# Autodesk Inventor assembly: finalassy
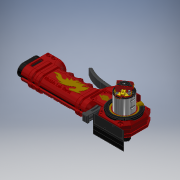
[picture p0: Inventor's stored thumbnail of the model, 180x180]
Saved by Autodesk Inventor 2018 (Build 220112000, 112)
## iProperties
Created: 2019-02-22
Part Number: finalassy
Material: 一般
Document SubType Name: Assembly
Designer: ku_sk
Author: ku_sk
## Documents named in this file (22)
- D:\Inventor\BayBladeLauncher\finalassy.iam
- D:\Inventor\BayBladeLauncher\parts\battery.ipt
- D:\Inventor\BayBladeLauncher\parts\brake.ipt
- D:\Inventor\BayBladeLauncher\parts\bay conect.ipt
- D:\Inventor\BayBladeLauncher\parts\bearing.ipt
- D:\Inventor\BayBladeLauncher\parts\bar.ipt
- D:\Inventor\BayBladeLauncher\parts\topcover.ipt
- D:\Inventor\BayBladeLauncher\parts\bar2.ipt
- D:\Inventor\BayBladeLauncher\parts\joint.ipt
- D:\Inventor\BayBladeLauncher\parts\switch.ipt
- D:\Inventor\BayBladeLauncher\parts\cover.ipt
- D:\Inventor\BayBladeLauncher\parts\ring.ipt
- D:\Inventor\BayBladeLauncher\parts\circuitcover.ipt
- D:\Inventor\BayBladeLauncher\parts\circuitcover1.ipt
- D:\Inventor\BayBladeLauncher\parts\gear.ipt
- D:\Inventor\BayBladeLauncher\parts\dragon.ipt
- D:\Inventor\BayBladeLauncher\parts\dragon_MIR.ipt
- D:\Inventor\BayBladeLauncher\parts\skyrimlogo2_1_9.ipt
- D:\Inventor\BayBladeLauncher\parts\pushbar.ipt
- D:\Inventor\BayBladeLauncher\reedy_540_rc_motor-1.snapshot.2\motor.iam
- D:\Inventor\BayBladeLauncher\parts\undercover1.ipt
- D:\Inventor\BayBladeLauncher\parts\undercover2.ipt
## Components (24 placed, 21 different names)
1. battery:1
2. bay conect:1 — メイト:8, メイト:9, メイト:10, メイト:19, フラッシュ:2
3. gear:1 — メイト:40, フラッシュ:2
4. bearing:1 — メイト:8, メイト:9, メイト:20
5. bar:1 — メイト:10, メイト:17, メイト:21, メイト:23, メイト:26
6. topcover:1 — メイト:28, メイト:29, メイト:30, メイト:31, メイト:32, メイト:40, メイト:49, 角度:1, メイト:50, メイト:53, メイト:54, メイト:55
7. bar2:1 — メイト:19, メイト:20, メイト:21
8. joint:1 — メイト:23, メイト:24, メイト:25, メイト:26
9. switch:1 — メイト:24, メイト:25, メイト:51, フラッシュ:4, メイト:52
10. cover:1 — メイト:30, メイト:31, メイト:32
11. ring:1 — メイト:28, メイト:29
12. circuitcover:1 — メイト:36, メイト:37, メイト:38, メイト:39
13. circuitcover1:1 — メイト:36, メイト:37, メイト:38, メイト:39
14. dragon:1
15. dragon_MIR:1
16. skyrimlogo2_1_9:1 — メイト:49, 角度:1, メイト:50
17. pushbar:1 — メイト:51, フラッシュ:4, メイト:52
18. motor:1 [sub-assembly] — メイト:53, メイト:54, メイト:55
19. undercover1:1 — メイト:56, メイト:57, メイト:58, メイト:59, メイト:60, メイト:61, メイト:62, メイト:63, メイト:64
20. undercover2:1 — メイト:56, メイト:57, メイト:58, メイト:59, メイト:60, メイト:61
21. brake:1 — メイト:17
22. brake:2
23. brake:3
24. brake:4
## Component patterns: (4 elements, first: brake:1)
## Relationships (40: Mate 37, Flush 2, Angle 1)
- メイト:8 [Mate]: bay conect:1 ↔ bearing:1
- メイト:9 [Mate]: bay conect:1 ↔ bearing:1
- メイト:10 [Mate]: bay conect:1 ↔ bar:1
- メイト:17 [Mate]: bar:1 ↔ brake:1
- メイト:19 [Mate]: bay conect:1 ↔ bar2:1
- メイト:20 [Mate]: bearing:1 ↔ bar2:1
- メイト:21 [Mate]: bar:1 ↔ bar2:1
- メイト:23 [Mate]: bar:1 ↔ joint:1
- メイト:24 [Mate]: joint:1 ↔ switch:1
- メイト:25 [Mate] (0.25 mm): joint:1 ↔ switch:1
- メイト:26 [Mate]: bar:1 ↔ joint:1
- メイト:28 [Mate]: topcover:1 ↔ ring:1
- メイト:29 [Mate]: topcover:1 ↔ ring:1
- メイト:30 [Mate]: topcover:1 ↔ cover:1
- メイト:31 [Mate]: topcover:1 ↔ cover:1
- メイト:32 [Mate]: topcover:1 ↔ cover:1
- メイト:36 [Mate]: circuitcover:1 ↔ circuitcover1:1
- メイト:37 [Mate]: circuitcover:1 ↔ circuitcover1:1
- メイト:38 [Mate]: circuitcover:1 ↔ circuitcover1:1
- メイト:39 [Mate]: circuitcover:1 ↔ circuitcover1:1
- メイト:40 [Mate]: gear:1 ↔ topcover:1
- フラッシュ:2 [Flush]: bay conect:1 ↔ gear:1
- メイト:49 [Mate]: topcover:1 ↔ skyrimlogo2_1_9:1
- 角度:1 [Angle] (26.37 deg): topcover:1 ↔ skyrimlogo2_1_9:1
- メイト:50 [Mate]: topcover:1 ↔ skyrimlogo2_1_9:1
- メイト:51 [Mate]: switch:1 ↔ pushbar:1
- フラッシュ:4 [Flush]: switch:1 ↔ pushbar:1
- メイト:52 [Mate]: switch:1 ↔ pushbar:1
- メイト:53 [Mate]: topcover:1 ↔ motor:1
- メイト:54 [Mate]: topcover:1 ↔ motor:1
- メイト:55 [Mate]: topcover:1 ↔ motor:1
- メイト:56 [Mate]: undercover1:1 ↔ undercover2:1
- メイト:57 [Mate]: undercover1:1 ↔ undercover2:1
- メイト:58 [Mate]: undercover1:1 ↔ undercover2:1
- メイト:59 [Mate]: undercover1:1 ↔ undercover2:1
- メイト:60 [Mate]: undercover1:1 ↔ undercover2:1
- メイト:61 [Mate]: undercover1:1 ↔ undercover2:1
- メイト:62 [Mate]: undercover1:1
- メイト:63 [Mate]: undercover1:1
- メイト:64 [Mate]: undercover1:1
